# Autodesk Inventor assembly: Pen Holder Assembly
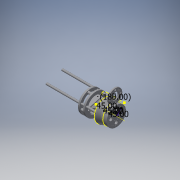
[picture p0: Inventor's stored thumbnail of the model, 180x180]
Saved by Autodesk Inventor 2019 (Build 230136000, 136)
## iProperties
Created: 2019-06-10
Part Number: Pen Holder Assembly
Document SubType Name: Assembly
Designer: Matthew XPS
Author: Matthew XPS
## Documents named in this file (7)
- G:\My Drive\Documents\Human Robot Interaction Lab\Projects\2019-06 Adept Viper Robot Arm\Pen  Holder\Pen Holder Assembly.iam
- G:\My Drive\Documents\Human Robot Interaction Lab\Projects\2019-06 Adept Viper Robot Arm\Pen  Holder\Clamp Plate.ipt
- G:\My Drive\Documents\Human Robot Interaction Lab\Projects\2019-06 Adept Viper Robot Arm\Pen  Holder\New Interface.ipt
- G:\My Drive\Documents\Human Robot Interaction Lab\Projects\2019-06 Adept Viper Robot Arm\Pen  Holder\Pen Holder Interface.ipt
- G:\My Drive\Documents\Human Robot Interaction Lab\Projects\2019-06 Adept Viper Robot Arm\Pen  Holder\Pen Main Piece.ipt
- G:\My Drive\Documents\Human Robot Interaction Lab\Projects\2019-06 Adept Viper Robot Arm\Pen  Holder\Robot Flange.ipt
- G:\My Drive\Documents\Human Robot Interaction Lab\Projects\2019-06 Adept Viper Robot Arm\Pen  Holder\6mm rod.ipt
## Components (8 placed, 6 different names)
1. Clamp Plate:1 — Rotational:1
2. New Interface:1 — Rigid:1, Rigid:2, Rotational:2, Rotational:3
3. Pen Holder Interface:1 — Rigid:1
4. Pen Main Piece:1 — Rotational:1, Mate:1, Mate:2
5. Robot Flange:1
6. 6mm rod:1 — Rigid:2, Mate:1
7. 6mm rod:2 — Rotational:2
8. 6mm rod:3 — Rotational:3, Mate:2
## Relationships (7: RevoluteJoint 3, WeldJoint 2, Mate 2)
- Rigid:1 [WeldJoint]: New Interface:1 ↔ Pen Holder Interface:1
- Rotational:1 [RevoluteJoint] (-0.5 mm): Clamp Plate:1 ↔ Pen Main Piece:1
- Rigid:2 [WeldJoint]: New Interface:1 ↔ 6mm rod:1
- Rotational:2 [RevoluteJoint]: New Interface:1 ↔ 6mm rod:2
- Rotational:3 [RevoluteJoint]: New Interface:1 ↔ 6mm rod:3
- Mate:1: Pen Main Piece:1 ↔ 6mm rod:1
- Mate:2: Pen Main Piece:1 ↔ 6mm rod:3
